# Autodesk Inventor assembly: HoodAssembled
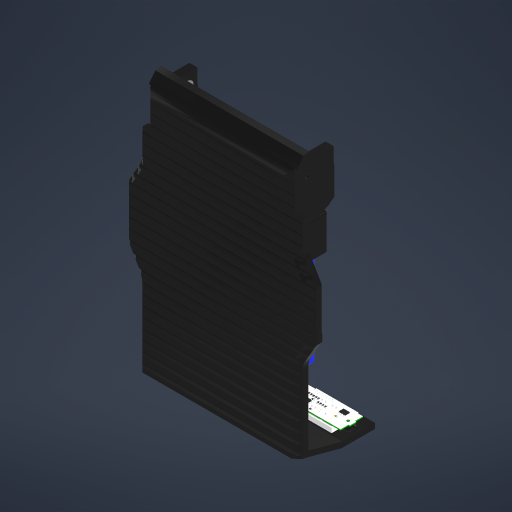
[picture p0: Inventor's stored thumbnail of the model, 512x512]
Saved by Autodesk Inventor 2023 (Build 270158000, 158)
## iProperties
Created: 2023-09-27
Part Number: HoodAssembled
Document SubType Name: Assembly
Designer: khrip
Author: khrip
## Documents named in this file (11)
- C:\GitHub\Botik\HoodAssembled.iam
- C:\GitHub\Botik\hood.ipt
- C:\GitHub\Botik\Magnet.ipt
- C:\Users\khrip\Documents\Inventor\Content Center Files\R2023\ru-RU\DIN 934\DIN 934 - M3 x 0,5.ipt
- C:\GitHub\Botik\BackBracket.ipt
- C:\GitHub\Botik\battery.ipt
- C:\GitHub\Botik\FrontBracket.ipt
- C:\Users\khrip\OneDrive\Документы\Inventor\Content Center Files\R2023\ru-RU\GOST 17475-80 (2)\Винт 2.M3-6gx8 ГОСТ 17475-80.ipt
- C:\Users\khrip\OneDrive\Документы\Inventor\Content Center Files\R2023\ru-RU\DIN 912\DIN 912 - M3 x 0,5 x 12 x 10,75.ipt
- C:\GitHub\Botik\Boards\Battery Level Indicator Module 1S-8S\STP\Battery Level Indicator Module 1S-8S.iam
- C:\GitHub\Botik\Switch\Wippschalter Rund - BG LED.iam
## Components (22 placed, 10 different names)
1. hood:1 — Совмещение:1, Совмещение:2, Заподлицо:1, Заподлицо:2, Совмещение:3, Совмещение:4, Заподлицо:3, Заподлицо:4, Вставка:1, Вставка:2, Вставка:3, Вставка:4, Вставка:5, Вставка:6, Угол:1, Угол:2, Угол:3, Угол:4, Угол:5, Угол:6, Совмещение:7, Совмещение:8, Совмещение:11, Совмещение:18, Совмещение:20, Заподлицо:5, Совмещение:21, Совмещение:22, Совмещение:23, Угол:8, Совмещение:24
2. Magnet:1 — Совмещение:1, Заподлицо:2
3. Magnet:2 — Совмещение:2, Заподлицо:1
4. Magnet:3 — Совмещение:3, Заподлицо:4
5. Magnet:4 — Совмещение:4, Заподлицо:3
6. DIN 934 - заменено на DIN EN 24032/28673/28674 M3:1 — Вставка:1, Угол:3, Совмещение:12
7. DIN 934 - заменено на DIN EN 24032/28673/28674 M3:2 — Вставка:2, Угол:6
8. DIN 934 - заменено на DIN EN 24032/28673/28674 M3:3 — Вставка:3, Угол:4, Совмещение:5
9. DIN 934 - заменено на DIN EN 24032/28673/28674 M3:4 — Вставка:4, Угол:5, Совмещение:6
10. DIN 934 - заменено на DIN EN 24032/28673/28674 M3:5 — Вставка:5, Угол:1, Совмещение:17
11. DIN 934 - заменено на DIN EN 24032/28673/28674 M3:6 — Вставка:6, Угол:2, Совмещение:19
12. BackBracket:1 — Совмещение:5, Совмещение:6, Совмещение:7, Совмещение:9, Совмещение:10, Угол:7, Совмещение:13, Совмещение:14, Совмещение:15
13. battery:1 — Совмещение:8, Совмещение:9, Совмещение:10
14. FrontBracket:1 — Совмещение:11, Совмещение:12, Угол:7, Совмещение:16
15. Винт 2 ГОСТ 17475-80 M3 x 8:1 — Совмещение:13
16. Винт 2 ГОСТ 17475-80 M3 x 8:2 — Совмещение:14
17. Винт 2 ГОСТ 17475-80 M3 x 8:3 — Совмещение:15
18. Винт 2 ГОСТ 17475-80 M3 x 8:4 — Совмещение:16
19. DIN 912 - заменено на DIN EN ISO 4762 M3 x 12:1 — Совмещение:17, Совмещение:18
20. DIN 912 - заменено на DIN EN ISO 4762 M3 x 12:2 — Совмещение:19, Совмещение:20
21. Battery Level Indicator Module 1S-8S:1 [sub-assembly] — Заподлицо:5, Совмещение:21, Совмещение:22
22. Wippschalter Rund - BG LED:1 [sub-assembly] — Совмещение:23, Угол:8, Совмещение:24
## Relationships (43: Mate 24, Angle 8, Insert 6, Flush 5)
- Совмещение:1 [Mate]: hood:1 ↔ Magnet:1
- Совмещение:2 [Mate]: hood:1 ↔ Magnet:2
- Заподлицо:1 [Flush]: hood:1 ↔ Magnet:2
- Заподлицо:2 [Flush]: hood:1 ↔ Magnet:1
- Совмещение:3 [Mate]: hood:1 ↔ Magnet:3
- Совмещение:4 [Mate]: hood:1 ↔ Magnet:4
- Заподлицо:3 [Flush]: hood:1 ↔ Magnet:4
- Заподлицо:4 [Flush]: hood:1 ↔ Magnet:3
- Вставка:1 [Insert]: hood:1 ↔ DIN 934 - заменено на DIN EN 24032/28673/28674 M3:1
- Вставка:2 [Insert]: hood:1 ↔ DIN 934 - заменено на DIN EN 24032/28673/28674 M3:2
- Вставка:3 [Insert]: hood:1 ↔ DIN 934 - заменено на DIN EN 24032/28673/28674 M3:3
- Вставка:4 [Insert]: hood:1 ↔ DIN 934 - заменено на DIN EN 24032/28673/28674 M3:4
- Вставка:5 [Insert]: hood:1 ↔ DIN 934 - заменено на DIN EN 24032/28673/28674 M3:5
- Вставка:6 [Insert]: hood:1 ↔ DIN 934 - заменено на DIN EN 24032/28673/28674 M3:6
- Угол:1 [Angle] (0 deg): hood:1 ↔ DIN 934 - заменено на DIN EN 24032/28673/28674 M3:5
- Угол:2 [Angle] (0 deg): hood:1 ↔ DIN 934 - заменено на DIN EN 24032/28673/28674 M3:6
- Угол:3 [Angle] (0 deg): hood:1 ↔ DIN 934 - заменено на DIN EN 24032/28673/28674 M3:1
- Угол:4 [Angle] (0 deg): hood:1 ↔ DIN 934 - заменено на DIN EN 24032/28673/28674 M3:3
- Угол:5 [Angle] (0 deg): hood:1 ↔ DIN 934 - заменено на DIN EN 24032/28673/28674 M3:4
- Угол:6 [Angle] (0 deg): hood:1 ↔ DIN 934 - заменено на DIN EN 24032/28673/28674 M3:2
- Совмещение:5 [Mate]: DIN 934 - заменено на DIN EN 24032/28673/28674 M3:3 ↔ BackBracket:1
- Совмещение:6 [Mate]: DIN 934 - заменено на DIN EN 24032/28673/28674 M3:4 ↔ BackBracket:1
- Совмещение:7 [Mate]: hood:1 ↔ BackBracket:1
- Совмещение:8 [Mate]: hood:1 ↔ battery:1
- Совмещение:9 [Mate] (1 mm): BackBracket:1 ↔ battery:1
- Совмещение:10 [Mate] (1 mm): BackBracket:1 ↔ battery:1
- Совмещение:11 [Mate]: hood:1 ↔ FrontBracket:1
- Совмещение:12 [Mate]: DIN 934 - заменено на DIN EN 24032/28673/28674 M3:1 ↔ FrontBracket:1
- Угол:7 [Angle] (0 deg): BackBracket:1 ↔ FrontBracket:1
- Совмещение:13 [Mate]: BackBracket:1 ↔ Винт 2 ГОСТ 17475-80 M3 x 8:1
- Совмещение:14 [Mate]: BackBracket:1 ↔ Винт 2 ГОСТ 17475-80 M3 x 8:2
- Совмещение:15 [Mate]: BackBracket:1 ↔ Винт 2 ГОСТ 17475-80 M3 x 8:3
- Совмещение:16 [Mate]: FrontBracket:1 ↔ Винт 2 ГОСТ 17475-80 M3 x 8:4
- Совмещение:17 [Mate]: DIN 934 - заменено на DIN EN 24032/28673/28674 M3:5 ↔ DIN 912 - заменено на DIN EN ISO 4762 M3 x 12:1
- Совмещение:18 [Mate]: hood:1 ↔ DIN 912 - заменено на DIN EN ISO 4762 M3 x 12:1
- Совмещение:19 [Mate]: DIN 934 - заменено на DIN EN 24032/28673/28674 M3:6 ↔ DIN 912 - заменено на DIN EN ISO 4762 M3 x 12:2
- Совмещение:20 [Mate]: hood:1 ↔ DIN 912 - заменено на DIN EN ISO 4762 M3 x 12:2
- Заподлицо:5 [Flush]: hood:1 ↔ Battery Level Indicator Module 1S-8S:1
- Совмещение:21 [Mate] (2.5 mm): hood:1 ↔ Battery Level Indicator Module 1S-8S:1
- Совмещение:22 [Mate] (10 mm): hood:1 ↔ Battery Level Indicator Module 1S-8S:1
- Совмещение:23 [Mate]: hood:1 ↔ Wippschalter Rund - BG LED:1
- Угол:8 [Angle] (180 deg): hood:1 ↔ Wippschalter Rund - BG LED:1
- Совмещение:24 [Mate]: hood:1 ↔ Wippschalter Rund - BG LED:1
